# Autodesk Inventor assembly: Chamber_assembly_vers_5
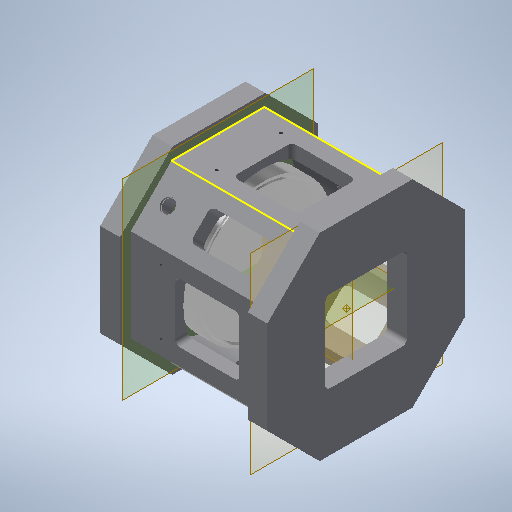
[picture p0: Inventor's stored thumbnail of the model, 512x512]
Saved by Autodesk Inventor 2025.4 (Build 294407000, 407)
## iProperties
Created: 2012-06-12
Part Number: Chamber_assembly_vers_5
Document SubType Name: Assembly
Designer: Breckenridge2 User
Author: Breckenridge2 User
## Documents named in this file (5)
- C:\Users\zboichykb\Documents\ResearchLocal\autodesk plasma chamber\Kuda_Topf_3D\Chamber_assembly_vers_5.iam
- C:\Users\zboichykb\Documents\ResearchLocal\autodesk plasma chamber\Kuda_Topf_3D\Chamber_wall_NEW_v_4.ipt
- C:\Users\zboichykb\Documents\ResearchLocal\autodesk plasma chamber\Kuda_Topf_3D\Electrode_assembly_v6.iam
- C:\Users\zboichykb\Documents\ResearchLocal\autodesk plasma chamber\Kuda_Topf_3D\chamber_top.ipt
- C:\Users\zboichykb\Documents\ResearchLocal\autodesk plasma chamber\Kuda_Topf_3D\chamber_base.ipt
## Components (4 placed, 4 different names)
1. Chamber_wall_NEW_v_4:1 — Insert:1, Insert:2, Insert:3
2. Electrode_assembly_v6:1 [sub-assembly] — Insert:1, Insert:2, Insert:3
3. chamber_top:1
4. chamber_base:1
## Relationships (3: Insert 3)
- Insert:1: Chamber_wall_NEW_v_4:1 ↔ Electrode_assembly_v6:1
- Insert:2: Chamber_wall_NEW_v_4:1 ↔ Electrode_assembly_v6:1
- Insert:3: Chamber_wall_NEW_v_4:1 ↔ Electrode_assembly_v6:1
